# Autodesk Inventor assembly: BAS_DTON
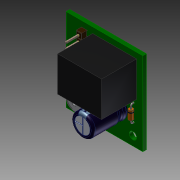
[picture p0: Inventor's stored thumbnail of the model, 180x180]
Saved by Autodesk Inventor 2013 (Build 170138000, 138)
## iProperties
Created: 2021-03-01
Part Number: BAS_DTON
Document SubType Name: Assembly
Designer: Fede
Translation Standard: STEP AP214IS
FileName: Open CASCADE Shape Model
PreProcessor: Open CASCADE 6.2
PostProcessor: Build: 138, Release: 2013 RTM - Date: Thu 03/01/2012
Sent Units: millimeter
Uncertainty: 0.0002
Author: Fede
## Documents named in this file (14)
- C:\0000 FEDE\16GB\0000 INTERIOR\DE_TMP_BAS\BAS_DTON - demora conexion al energizar\DTON_MANUAL\img\INVENTOR\BAS_DTON_PIN - SIN R\BAS_DTON_PIN - SIN R.iam
- C:\0000 FEDE\16GB\0000 INTERIOR\DE_TMP_BAS\BAS_DTON - demora conexion al energizar\DTON_MANUAL\img\INVENTOR\BAS_DTON_PIN - SIN R\Board.ipt
- C:\0000 FEDE\16GB\0000 INTERIOR\DE_TMP_BAS\BAS_DTON - demora conexion al energizar\DTON_MANUAL\img\INVENTOR\BAS_DTON_PIN - SIN R\D3.iam
- C:\0000 FEDE\16GB\0000 INTERIOR\DE_TMP_BAS\BAS_DTON - demora conexion al energizar\DTON_MANUAL\img\INVENTOR\BAS_DTON_PIN - SIN R\R5.iam
- C:\0000 FEDE\16GB\0000 INTERIOR\DE_TMP_BAS\BAS_DTON - demora conexion al energizar\DTON_MANUAL\img\INVENTOR\BAS_DTON_PIN - SIN R\K1.iam
- C:\0000 FEDE\16GB\0000 INTERIOR\DE_TMP_BAS\BAS_DTON - demora conexion al energizar\DTON_MANUAL\img\INVENTOR\BAS_DTON_PIN - SIN R\R1.iam
- C:\0000 FEDE\16GB\0000 INTERIOR\DE_TMP_BAS\BAS_DTON - demora conexion al energizar\DTON_MANUAL\img\INVENTOR\BAS_DTON_PIN - SIN R\C3.iam
- C:\0000 FEDE\16GB\0000 INTERIOR\DE_TMP_BAS\BAS_DTON - demora conexion al energizar\DTON_MANUAL\img\INVENTOR\BAS_DTON_PIN - SIN R\Q1.iam
- C:\0000 FEDE\16GB\0000 INTERIOR\DE_TMP_BAS\BAS_DTON - demora conexion al energizar\DTON_MANUAL\img\INVENTOR\BAS_DTON_PIN - SIN R\R7.iam
- C:\0000 FEDE\16GB\0000 INTERIOR\DE_TMP_BAS\BAS_DTON - demora conexion al energizar\DTON_MANUAL\img\INVENTOR\BAS_DTON_PIN - SIN R\D2.iam
- C:\0000 FEDE\16GB\0000 INTERIOR\DE_TMP_BAS\BAS_DTON - demora conexion al energizar\DTON_MANUAL\img\INVENTOR\BAS_DTON_PIN - SIN R\R8.iam
- C:\0000 FEDE\16GB\0000 INTERIOR\DE_TMP_BAS\BAS_DTON - demora conexion al energizar\DTON_MANUAL\img\INVENTOR\BAS_DTON_PIN - SIN R\R2.iam
- C:\0000 FEDE\16GB\0000 INTERIOR\DE_TMP_BAS\BAS_DTON - demora conexion al energizar\DTON_MANUAL\img\INVENTOR\BAS_DTON_PIN - SIN R\Free-Models.iam
- C:\0000 FEDE\16GB\0000 INTERIOR\DE_TMP_BAS\BAS_DTON - demora conexion al energizar\DTON_MANUAL\img\INVENTOR\BAS_DTON_PIN - SIN R\pin1x1.iam
## Components (17 placed, 13 different names)
1. Board:1 — Mate:1
2. D3:1 [sub-assembly]
3. R5:1 [sub-assembly]
4. K1:1 [sub-assembly]
5. R1:1 [sub-assembly]
6. C3:1 [sub-assembly]
7. Q1:1 [sub-assembly]
8. R7:1 [sub-assembly]
9. D2:1 [sub-assembly]
10. R8:1 [sub-assembly]
11. R2:1 [sub-assembly]
12. Free-Models:1 [sub-assembly] — Mate:2, Flush:1
13. pin1x1:1 [sub-assembly] — Mate:1, Mate:2, Flush:1
14. pin1x1:2 [sub-assembly]
15. pin1x1:3 [sub-assembly]
16. pin1x1:4 [sub-assembly]
17. pin1x1:5 [sub-assembly]
## Component patterns: (5 elements, first: pin1x1:1)
## Relationships (3: Mate 2, Flush 1)
- Mate:1: Board:1 ↔ pin1x1:1
- Mate:2: Free-Models:1 ↔ pin1x1:1
- Flush:1: Free-Models:1 ↔ pin1x1:1
